# Autodesk Inventor assembly: LoadCell_unit
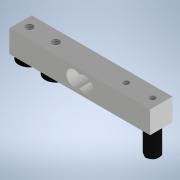
[picture p0: Inventor's stored thumbnail of the model, 180x180]
Saved by Autodesk Inventor 2022.3 (Build 263350000, 350)
## iProperties
Created: 2023-04-23
Part Number: LoadCell_unit
Document SubType Name: Assembly
Designer: Masato Kubotera
Author: Masato Kubotera
## Documents named in this file (4)
- C:\Users\Masato\OneDrive - Chiba Institute of Technology\CIT Brains\RoboCup2023\GitHub Repository\SUSTAINA-OP\LowerBody\Foot\LoadCell_unit.iam
- C:\Users\Masato\OneDrive - Chiba Institute of Technology\CIT Brains\RoboCup2023\GitHub Repository\SUSTAINA-OP\ReadyMade\ElectronicComponents\SC133-20kg.ipt
- C:\Users\Masato\OneDrive - Chiba Institute of Technology\CIT Brains\RoboCup2023\GitHub Repository\SUSTAINA-OP\ReadyMade\Spacer\BSL-415BE.ipt
- C:\Users\Masato\OneDrive - Chiba Institute of Technology\CIT Brains\RoboCup2023\GitHub Repository\SUSTAINA-OP\ReadyMade\Washer\UUW-0512-30BH.ipt
## Components (4 placed, 3 different names)
1. SC133-20kg:1 — フラッシュ:1, フラッシュ:2, フラッシュ:3, 挿入:1, 角度:1, 挿入:2, 挿入:3
2. BSL-415BE:1 — 挿入:1, 角度:1
3. UUW-0512-30BH:1 — 挿入:2
4. UUW-0512-30BH:2 — 挿入:3
## Relationships (7: Flush 3, Insert 3, Angle 1)
- フラッシュ:1 [Flush]: SC133-20kg:1
- フラッシュ:2 [Flush]: SC133-20kg:1
- フラッシュ:3 [Flush]: SC133-20kg:1
- 挿入:1 [Insert]: SC133-20kg:1 ↔ BSL-415BE:1
- 角度:1 [Angle] (0 deg): SC133-20kg:1 ↔ BSL-415BE:1
- 挿入:2 [Insert]: SC133-20kg:1 ↔ UUW-0512-30BH:1
- 挿入:3 [Insert]: SC133-20kg:1 ↔ UUW-0512-30BH:2
